# Autodesk Inventor assembly: moving_block_with_connector
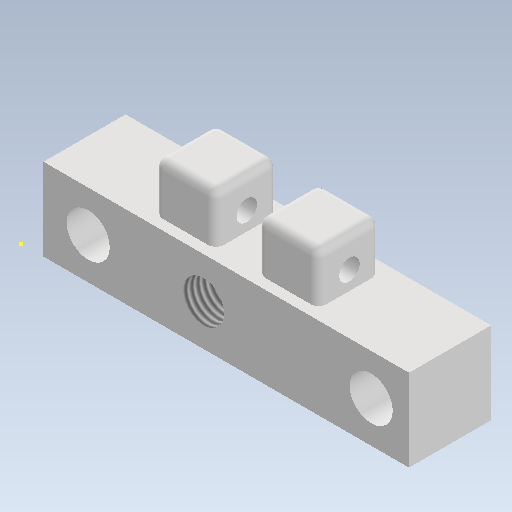
[picture p0: Inventor's stored thumbnail of the model, 512x512]
Saved by Autodesk Inventor 2021 (Build 250183000, 183)
## iProperties
Created: 2021-02-06
Part Number: moving_block_with_connector
Document SubType Name: Assembly
Designer: chris
Mass: 35.2018 g
Surface Area: 119.002 cm^2
Volume: 35.2018 cm^3
Density: 1 g/cm^3
Author: chris
## Documents named in this file (3)
- C:\Users\chris\Desktop\Project 3 Device\moving_block_with_connector.iam
- C:\Users\chris\Desktop\Project 3 Device\moving_block.ipt
- C:\Users\chris\Desktop\Project 3 Device\Connector.ipt
## Components (3 placed, 2 different names)
1. moving_block:1 — Mate:2, Flush:2, Flush:3, Mate:3
2. Connector:1 — Mate:1, Mate:2, Flush:1, Flush:2, Flush:3
3. Connector:2 — Mate:1, Flush:1, Mate:3
## Relationships (6: Mate 3, Flush 3)
- Mate:1 (10 mm): Connector:1 ↔ Connector:2
- Mate:2: moving_block:1 ↔ Connector:1
- Flush:1: Connector:1 ↔ Connector:2
- Flush:2 (-24.5 mm): moving_block:1 ↔ Connector:1
- Flush:3 (2.5 mm): moving_block:1 ↔ Connector:1
- Mate:3: moving_block:1 ↔ Connector:2
